# Autodesk Inventor assembly: Buse E3D V6
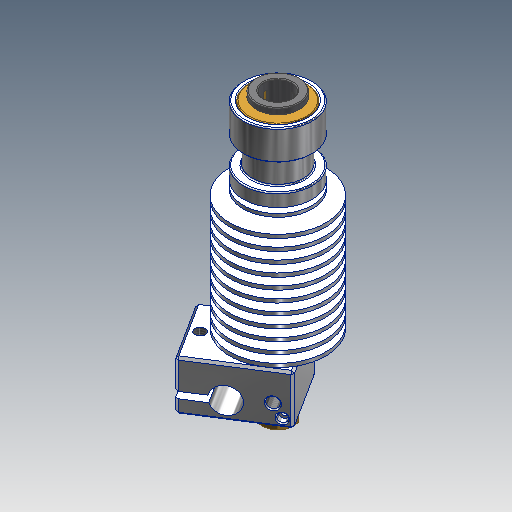
[picture p0: Inventor's stored thumbnail of the model, 512x512]
Saved by Autodesk Inventor 2017 (Build 210142000, 142)
## iProperties
Company: FABLAB Frenchmakers
Part Number: Buse E3D V6
Material: Générique
Document SubType Name: Assembly
Designer: FABLAB Frenchmakers
Mass: 33.155 g
Surface Area: 144.774 cm^2
Volume: 10.3764 cm^3
Density: 3.19523 g/cm^3
Stock Number: 1420-02-20
Project: 1420 Vauban 3D XL
Catalog Web Link: http://frenchmakers.com/
## Documents named in this file (7)
- W:\Professionnel\Conception FABLAB\1420-Vauban 3D XL\1420-02 Tete\Buse_E3D_V6\1420-02-20 Buse E3d V6.iam
- W:\Professionnel\Conception FABLAB\1420-Vauban 3D XL\1420-02 Tete\Buse_E3D_V6\1420-02-24 Base.ipt
- W:\Professionnel\Conception FABLAB\1420-Vauban 3D XL\1420-02 Tete\Buse_E3D_V6\1420-02-23 Vis de raccord.ipt
- W:\Professionnel\Conception FABLAB\1420-Vauban 3D XL\1420-02 Tete\Buse_E3D_V6\1420-02-22 Bloque de chauffe.ipt
- W:\Professionnel\Conception FABLAB\1420-Vauban 3D XL\1420-02 Tete\Buse_E3D_V6\1420-02-21 Buse 04.ipt
- W:\Professionnel\Conception FABLAB\1420-Vauban 3D XL\1420-02 Tete\Buse_E3D_V6\1420-02-25 Bague.ipt
- W:\Professionnel\Conception FABLAB\1420-Vauban 3D XL\1420-02 Tete\Buse_E3D_V6\1420-02-26 Clip pneumatique.ipt
## Components (6 placed, 6 different names)
1. 1420-02-24 Base:1 — Affleurement:1, Affleurement:2, Affleurement:3, Placage:1, Placage:2, Placage:7, Affleurement:5
2. 1420-02-23 Vis de raccord:1 — Placage:1, Placage:2, Placage:3, Affleurement:4, Placage:6
3. 1420-02-22 Bloque de chauffe:1 — Placage:3, Affleurement:4, Placage:4
4. 1420-02-21 Buse 04:1 — Placage:4, Placage:6
5. 1420-02-25 Bague:1 — Placage:7, Affleurement:5, Placage:8, Placage:9
6. 1420-02-26 Clip pneumatique:1 — Placage:8, Placage:9
## Relationships (13: Mate 8, Flush 5)
- Affleurement:1 [Flush]: 1420-02-24 Base:1
- Affleurement:2 [Flush]: 1420-02-24 Base:1
- Affleurement:3 [Flush]: 1420-02-24 Base:1
- Placage:1 [Mate]: 1420-02-24 Base:1 ↔ 1420-02-23 Vis de raccord:1
- Placage:2 [Mate]: 1420-02-24 Base:1 ↔ 1420-02-23 Vis de raccord:1
- Placage:3 [Mate]: 1420-02-23 Vis de raccord:1 ↔ 1420-02-22 Bloque de chauffe:1
- Affleurement:4 [Flush]: 1420-02-23 Vis de raccord:1 ↔ 1420-02-22 Bloque de chauffe:1
- Placage:4 [Mate]: 1420-02-22 Bloque de chauffe:1 ↔ 1420-02-21 Buse 04:1
- Placage:6 [Mate]: 1420-02-23 Vis de raccord:1 ↔ 1420-02-21 Buse 04:1
- Placage:7 [Mate]: 1420-02-24 Base:1 ↔ 1420-02-25 Bague:1
- Affleurement:5 [Flush]: 1420-02-24 Base:1 ↔ 1420-02-25 Bague:1
- Placage:8 [Mate]: 1420-02-25 Bague:1 ↔ 1420-02-26 Clip pneumatique:1
- Placage:9 [Mate] (0.5 mm): 1420-02-25 Bague:1 ↔ 1420-02-26 Clip pneumatique:1
